# Autodesk Inventor assembly: 右足アセンブリ
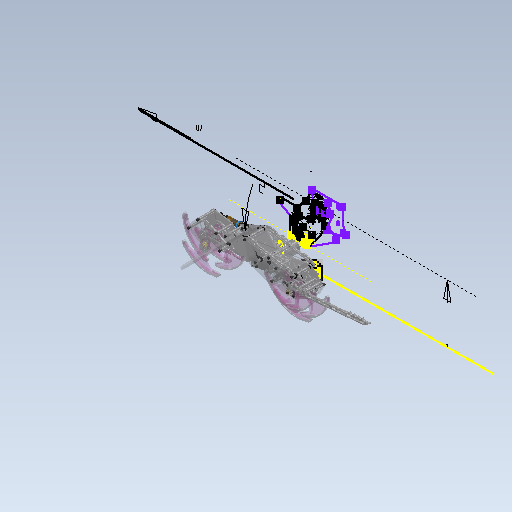
[picture p0: Inventor's stored thumbnail of the model, 512x512]
Saved by Autodesk Inventor 2020 (Build 240168000, 168)
## iProperties
Created: 2019-09-17
Part Number: 右足アセンブリ
Material: 一般
Document SubType Name: Assembly
Designer: tanjihayato
Mass: 847.137 g
Surface Area: 3618.61 cm^2
Volume: 359.726 cm^3
Density: 2.35495 g/cm^3
Author: tanjihayato
## Documents named in this file (54)
- \\Mac\Home\Documents\Inventor\2019お遊び機体\右足アセンブリ.iam
- \\Mac\Home\Documents\Inventor\2019お遊び機体\前足内フレーム.ipt
- \\Mac\Home\Documents\Inventor\2019お遊び機体\新型３クランクアセンブリ.iam
- \\Mac\Home\Documents\Inventor\2019お遊び機体\新型３脚最終段カム.ipt
- \\Mac\Home\Documents\Inventor\2019お遊び機体\スペーサ　m3-l35.ipt
- \\Mac\Home\Documents\Inventor\2019お遊び機体\新型３ヘッケン.ipt
- \\Mac\Home\Documents\Inventor\2019お遊び機体\新型３揺動節.ipt
- \\Mac\Home\Documents\Inventor\2019お遊び機体\線図.ipt
- \\Mac\Home\Documents\Inventor\2019お遊び機体\ギアトレイン.ipt
- \\Mac\Home\Documents\Inventor\2019お遊び機体\前足外フレーム.ipt
- \\Mac\Home\Documents\Inventor\2019お遊び機体\後ろ脚内フレーム.ipt
- \\Mac\Home\Documents\Inventor\2019お遊び機体\後ろ脚内フレーム２.ipt
- \\Mac\Home\Documents\Inventor\2019お遊び機体\新型３クランクアセンブリ_MIR.iam
- \\Mac\Home\Documents\Inventor\2019お遊び機体\新型３ヘッケン_MIR.ipt
- \\Mac\Home\Documents\Inventor\2019お遊び機体\新型３揺動節_MIR.ipt
- \\Mac\Home\Documents\Inventor\2019お遊び機体\後ろ脚外フレーム.ipt
- \\Mac\Home\Documents\Inventor\2019お遊び機体\前足ギアトレイン抑え.ipt
- \\Mac\Home\Documents\Inventor\2019お遊び機体\スペーサ　m3-l6.ipt
- \\Mac\Home\Documents\Inventor\2019お遊び機体\z28ギア(インベンター).ipt
- \\Mac\Home\Documents\Inventor\2019お遊び機体\z20ギア(インベンター).ipt
- \\Mac\Home\Documents\Inventor\2019お遊び機体\ベアリングフランジ6-12.ipt
- \\Mac\Home\Documents\Inventor\2019お遊び機体\z17ギア(インベンター).ipt
- \\Mac\Home\Documents\Inventor\2019お遊び機体\新型３脚最終段カム2.ipt
- \\Mac\Home\Documents\Inventor\2019お遊び機体\中間内フレーム2.ipt
- \\Mac\Home\Documents\Inventor\2019お遊び機体\サス軸抑え外.ipt
- \\Mac\Home\Documents\Inventor\2019お遊び機体\中間外フレーム2.ipt
- \\Mac\Home\Documents\Inventor\2019お遊び機体\タミヤダンパー1.iam
- \\Mac\Home\Documents\Inventor\2019お遊び機体\脚ゴム.ipt
- \\Mac\Home\Documents\Inventor\2019お遊び機体\歯車m0.5.z80.ipt
- \\Mac\Home\Documents\Inventor\2019お遊び機体\m2z10.ipt
- \\Mac\Home\Documents\Inventor\2019お遊び機体\中間フレーム内内.ipt
- \\Mac\Home\Documents\Inventor\2019お遊び機体\モーター(形だけ).ipt
- \\Mac\Home\Documents\Inventor\2019お遊び機体\脚モーターマウント.ipt
- \\Mac\Home\Documents\Inventor\2019お遊び機体\台形サスバー２.ipt
- \\Mac\Home\Documents\Inventor\2019お遊び機体\フランジブッシュ　d6-D8-l5-h12.ipt
- \\Mac\Home\Documents\Inventor\2019お遊び機体\スペーサ　m3-l45.ipt
- \\Mac\Home\Documents\Inventor\2019お遊び機体\台形サスバー板.ipt
- \\Mac\Home\Documents\Inventor\2019お遊び機体\台形サスカバー.ipt
- \\Mac\Home\Documents\Inventor\2019お遊び機体\カウンター短.ipt
- \\Mac\Home\Documents\Inventor\2019お遊び機体\ベアリングH　d6-D10-B3.ipt
- \\Mac\Home\Documents\Inventor\2019お遊び機体\スペーサ　m4-l35.ipt
- \\Mac\Home\Documents\Inventor\2019お遊び機体\スペーサ　m3-l14.ipt
- \\Mac\Home\Documents\Inventor\2019お遊び機体\キャップボルトM3×8.ipt
- \\Mac\Home\Documents\Inventor\2019お遊び機体\スペーサ　m3-l4.ipt
- \\Mac\Home\Documents\Inventor\2019お遊び機体\フランジブッシュ　d12-14-F20.ipt
- \\Mac\Home\Documents\Inventor\2019お遊び機体\オイレス　d12-D14-L3.ipt
- \\Mac\Home\Documents\Inventor\2019お遊び機体\キャップボルトM3×20.ipt
- \\Mac\Home\Documents\Inventor\2019お遊び機体\後ろ脚内内フレーム.ipt
- \\Mac\Home\Documents\Inventor\2019お遊び機体\ウイング土台.ipt
- \\Mac\Home\Documents\Inventor\2019お遊び機体\新型４ウイング.ipt
- \\Mac\Home\Documents\Inventor\2019お遊び機体\ウイング抑え.ipt
- \\Mac\Home\Documents\Inventor\2019お遊び機体\ねじ皿　m3-l8.ipt
- \\Mac\Home\Documents\Inventor\2019お遊び機体\新型４留め具.ipt
- \\Mac\Home\Documents\Inventor\2019お遊び機体\モーターマウントっぽい.ipt
## Components (192 placed, 53 different names)
1. 前足内フレーム:1 — 挿入:29, 挿入:32, 挿入:37, 挿入:127, 挿入:134, 挿入:135, 挿入:152, 挿入:181, 挿入:229, 挿入:230
2. 新型３クランクアセンブリ:1 [sub-assembly] — 挿入:1, メイト:1, 挿入:8, 挿入:9, 挿入:10, 挿入:11, 挿入:230
3. 新型３脚最終段カム:1 — 挿入:1, メイト:1, 挿入:62, メイト:44
4. スペーサ　m3-l35:2 — 挿入:29, 挿入:149
5. スペーサ　m3-l35:4 — メイト:2, メイト:3, メイト:4, メイト:5, 挿入:32, メイト:15
6. 新型３ヘッケン:1 — 挿入:11, 挿入:14, メイト:56, メイト:57, フラッシュ:2
7. 新型３ヘッケン:2 — 挿入:10, 挿入:13, メイト:60, メイト:61, フラッシュ:4
8. 新型３ヘッケン:3 — 挿入:9, 挿入:12, メイト:62, メイト:63, フラッシュ:5
9. 新型３ヘッケン:4 — 挿入:7, 挿入:8, メイト:58, メイト:59, フラッシュ:3
10. 新型３揺動節:1 — メイト:2, 挿入:7
11. 新型３揺動節:2 — メイト:3, 挿入:13
12. 新型３揺動節:3 — メイト:4, 挿入:12
13. 新型３揺動節:4 — メイト:5, 挿入:14
14. 線図:1 — メイト:91, メイト:92
15. ギアトレイン:1 — 挿入:15, 挿入:16, 挿入:17, 挿入:18, 挿入:19, 挿入:20, 挿入:154, 挿入:189
16. ギアトレイン:2 — 挿入:21, メイト:10, 挿入:37, 挿入:153, 挿入:187
17. スペーサ　m3-l6:3 — 挿入:17
18. スペーサ　m3-l6:2 — 挿入:20, メイト:10
19. スペーサ　m3-l6:5 — 挿入:19
20. スペーサ　m3-l6:1 — 挿入:16, 挿入:69
21. スペーサ　m3-l6:6 — 挿入:15, 挿入:21
22. スペーサ　m3-l6:4 — 挿入:18, 挿入:67
23. スペーサ　m3-l35:5 — メイト:55, 挿入:119
24. スペーサ　m3-l35:6
25. スペーサ　m3-l35:8 — メイト:53
26. 前足外フレーム:1 — メイト:15, 挿入:128, 挿入:136, メイト:84, 挿入:149, 挿入:165, 挿入:182, 挿入:226
27. 後ろ脚内フレーム:1 — 挿入:41, メイト:17, 挿入:71, 挿入:73, 挿入:76, 挿入:77, 挿入:188, 挿入:192, 挿入:193, 挿入:194, 挿入:195
28. 後ろ脚内フレーム２:1 — 挿入:41, メイト:17, 挿入:51, 挿入:52, 挿入:53, 挿入:54, 挿入:138, 挿入:139, 挿入:140, 挿入:155, 挿入:205, 挿入:227
29. 新型３クランクアセンブリ_MIR:1 [sub-assembly] — 挿入:43, 挿入:44, 挿入:45, 挿入:46, 挿入:55, メイト:18
30. 新型３ヘッケン_MIR:1 — 挿入:43, 挿入:50, メイト:66, メイト:67, フラッシュ:7
31. 新型３ヘッケン_MIR:2 — 挿入:44, 挿入:48, メイト:64, メイト:65, フラッシュ:6
32. 新型３ヘッケン_MIR:3 — 挿入:45, 挿入:49, メイト:68, メイト:69, フラッシュ:8
33. 新型３ヘッケン_MIR:4 — 挿入:46, 挿入:47, メイト:70, メイト:71, フラッシュ:9
34. 新型３揺動節_MIR:1 — 挿入:47, メイト:20
35. 新型３揺動節_MIR:3 — 挿入:49, メイト:21
36. 新型３揺動節_MIR:4 — 挿入:50, メイト:19
37. スペーサ　m3-l35:9 — 挿入:52, メイト:23
38. スペーサ　m3-l35:10 — 挿入:51
39. スペーサ　m3-l35:11 — 挿入:54, メイト:19, メイト:20, メイト:21, メイト:22, 挿入:57
40. スペーサ　m3-l35:12 — 挿入:53
41. 新型３脚最終段カム:2 — 挿入:55, メイト:18, 挿入:74, メイト:48, 挿入:227
42. 後ろ脚外フレーム:1 — 挿入:57, メイト:23, 挿入:141, 挿入:142, 挿入:143, 挿入:144, 挿入:225
43. 前足ギアトレイン抑え:1 — 挿入:151, 挿入:237, 挿入:238, 挿入:239, 挿入:240
44. スペーサ　m3-l14:1
45. スペーサ　m3-l14:2 — 挿入:237
46. スペーサ　m3-l14:3 — 挿入:229
47. 新型３脚最終段カム2:1 — 挿入:62, メイト:44, 挿入:63, メイト:45
48. z28ギア(インベンター):1 — 挿入:63, メイト:45, 挿入:64, メイト:47
49. 新型３脚最終段カム:4 — 挿入:65, メイト:46, メイト:100
50. 新型３脚最終段カム:5 — 挿入:64, 挿入:65, メイト:46, メイト:47
51. z20ギア(インベンター):1 — 挿入:66
52. ベアリングフランジ6-12:1 — 挿入:66, 挿入:67
53. z17ギア(インベンター):1 — 挿入:68
54. ベアリングフランジ6-12:2 — 挿入:68, 挿入:69
55. z17ギア(インベンター):2
56. ベアリングフランジ6-12:3 — 挿入:71
57. z20ギア(インベンター):2
58. ベアリングフランジ6-12:4 — 挿入:73
59. z28ギア(インベンター):2 — 挿入:75, メイト:49
60. 新型３脚最終段カム:6 — 挿入:74, メイト:48, 挿入:75, メイト:49
61. スペーサ　m3-l6:7 — 挿入:76
62. スペーサ　m3-l6:8 — 挿入:77
63. 中間内フレーム2:1 — 挿入:78, メイト:50, 挿入:94, 挿入:95, 挿入:96, 挿入:97, 挿入:98, 挿入:124, 挿入:147, 挿入:148, 挿入:217, 挿入:218, 挿入:221, 挿入:231, 挿入:232, 挿入:233, 挿入:234, 挿入:235, 挿入:236
64. サス軸抑え外:1 — 挿入:78, メイト:50, 挿入:198, 挿入:199, 挿入:200, 挿入:201
65. 中間外フレーム2:1 — メイト:53, 挿入:119, メイト:79, 挿入:120, 挿入:145, 挿入:146, 挿入:164, 挿入:213, メイト:88, 挿入:219, 挿入:220, メイト:91, メイト:92
66. スペーサ　m3-l4:2
67. スペーサ　m3-l4:1
68. スペーサ　m3-l4:3
69. タミヤダンパー1:1 [sub-assembly] — メイト:55, 挿入:118
70. 脚ゴム:1 — メイト:68, メイト:69, フラッシュ:8
71. 脚ゴム:2 — メイト:70, メイト:71, フラッシュ:9
72. 脚ゴム:3 — メイト:56, メイト:57, フラッシュ:2
73. 脚ゴム:4 — メイト:66, メイト:67, フラッシュ:7
74. 脚ゴム:5 — メイト:60, メイト:61, フラッシュ:4
75. 脚ゴム:6 — メイト:64, メイト:65, フラッシュ:6
76. 脚ゴム:7 — メイト:62, メイト:63, フラッシュ:5
77. 脚ゴム:8 — メイト:58, メイト:59, フラッシュ:3
78. 歯車m0.5.z80:1 — 挿入:102, 挿入:103, 挿入:104, 挿入:105, メイト:74
79. m2z10:1 — 挿入:94, 挿入:106, メイト:74
80. スペーサ　m3-l6:9 — 挿入:98, メイト:73, メイト:75
81. スペーサ　m3-l6:10 — 挿入:96
82. スペーサ　m3-l6:11 — 挿入:95
83. スペーサ　m3-l6:12 — 挿入:97, 挿入:99, 挿入:107
84. サス軸抑え外:2 — 挿入:99, メイト:73, 挿入:183, 挿入:184, 挿入:185, 挿入:186, 挿入:202, 挿入:203
85. スペーサ　m3-l6:13 — 挿入:105
86. スペーサ　m3-l6:14 — 挿入:104
87. スペーサ　m3-l6:15 — 挿入:103
88. スペーサ　m3-l6:16 — 挿入:102, 挿入:106
89. 中間フレーム内内:1 — 挿入:107, メイト:75, 挿入:172, 挿入:173, 挿入:208, 挿入:209, 挿入:210, 挿入:211
90. モーター(形だけ):1 — 挿入:242
91. モーター(形だけ):2 — 挿入:243
92. スペーサ　m3-l14:6 — 挿入:211, 挿入:212
93. スペーサ　m3-l14:4 — 挿入:209
94. スペーサ　m3-l14:5 — 挿入:210
95. スペーサ　m3-l14:7 — 挿入:208, メイト:87
96. 脚モーターマウント:1 — 挿入:166, 挿入:167, 挿入:168, 挿入:169, 挿入:212, メイト:93, メイト:94, メイト:95, メイト:96, メイト:97, メイト:98, 挿入:228
97. 台形サスバー２:1 — メイト:79, 挿入:121, 挿入:122, 挿入:123, 挿入:129, 挿入:130, メイト:83, 挿入:160
98. 台形サスバー２:2 — 挿入:118, メイト:81, フラッシュ:10, メイト:82, 挿入:137, メイト:85, 挿入:156, 挿入:157, 挿入:158, 挿入:159
99. フランジブッシュ　d6-D8-l5-h12:1 — 挿入:128, 挿入:150
100. フランジブッシュ　d6-D8-l5-h12:2 — 挿入:120
101. フランジブッシュ　d6-D8-l5-h12:3 — 挿入:127
102. フランジブッシュ　d6-D8-l5-h12:4 — 挿入:124, 挿入:137
103. スペーサ　m3-l45:1 — 挿入:121
104. スペーサ　m3-l45:2 — 挿入:122, メイト:85, 挿入:150
105. スペーサ　m3-l45:3 — 挿入:123
106. スペーサ　m3-l45:4 — 挿入:129
107. 台形サスバー板:1 — メイト:81, フラッシュ:10, メイト:82
108. 台形サスカバー:1 — 挿入:130, メイト:83, 挿入:161, 挿入:162, 挿入:163
109. カウンター短:1 — 挿入:136, メイト:84
110. ベアリングH　d6-D10-B3:1 — 挿入:225
111. ベアリングH　d6-D10-B3:2 — 挿入:226
112. スペーサ　m4-l35:1 — 挿入:135
113. スペーサ　m4-l35:2 — 挿入:134
114. キャップボルトM3×8:1 — 挿入:138
115. キャップボルトM3×8:2 — 挿入:139
116. キャップボルトM3×8:3 — 挿入:141
117. キャップボルトM3×8:4 — 挿入:144
118. キャップボルトM3×8:5 — 挿入:140
119. キャップボルトM3×8:6 — 挿入:145
120. キャップボルトM3×8:7 — 挿入:146
121. キャップボルトM3×8:8 — 挿入:143
122. キャップボルトM3×8:9 — 挿入:142
123. キャップボルトM3×8:10 — 挿入:147
124. キャップボルトM3×8:11 — 挿入:148
125. フランジブッシュ　d12-14-F20:1 — 挿入:151, メイト:100
126. フランジブッシュ　d12-14-F20:2 — 挿入:152
127. フランジブッシュ　d12-14-F20:3 — 挿入:155
128. オイレス　d12-D14-L3:1 — 挿入:153
129. オイレス　d12-D14-L3:2 — 挿入:154
130. キャップボルトM3×8:12 — 挿入:156
131. キャップボルトM3×8:13 — 挿入:157
132. キャップボルトM3×8:14 — 挿入:160
133. キャップボルトM3×8:15 — 挿入:159
134. キャップボルトM3×8:16 — 挿入:161
135. キャップボルトM3×8:17 — 挿入:162
136. キャップボルトM3×8:18 — 挿入:158
137. キャップボルトM3×8:19 — 挿入:163
138. キャップボルトM3×8:20 — 挿入:164
139. キャップボルトM3×8:21 — 挿入:166, メイト:87
140. キャップボルトM3×8:22 — 挿入:165
141. キャップボルトM3×8:23 — 挿入:167, 挿入:241
142. キャップボルトM3×8:24 — 挿入:168
143. キャップボルトM3×8:25 — 挿入:169, メイト:102
144. キャップボルトM3×8:26 — 挿入:236
145. キャップボルトM3×8:27 — 挿入:235
146. キャップボルトM3×8:30 — 挿入:172
147. キャップボルトM3×8:31 — 挿入:173
148. キャップボルトM3×20:1 — 挿入:239
149. キャップボルトM3×20:2 — 挿入:238
150. キャップボルトM3×20:3 — 挿入:240
151. キャップボルトM3×20:4 — 挿入:184
152. キャップボルトM3×20:5 — 挿入:183
153. キャップボルトM3×20:6 — 挿入:185
154. キャップボルトM3×20:7 — 挿入:186
155. キャップボルトM3×8:32 — 挿入:181
156. キャップボルトM3×8:33 — 挿入:182
157. スペーサ　m3-l4:4 — 挿入:187, 挿入:196, 挿入:199
158. スペーサ　m3-l4:5 — 挿入:188, 挿入:197, 挿入:198
159. スペーサ　m3-l4:6 — 挿入:189
160. キャップボルトM3×20:8 — 挿入:196
161. キャップボルトM3×20:9 — 挿入:197
162. スペーサ　m3-l6:17 — 挿入:195
163. スペーサ　m3-l6:18 — 挿入:194
164. スペーサ　m3-l6:19 — 挿入:193, 挿入:204
165. スペーサ　m3-l6:20 — 挿入:192, メイト:86
166. フランジブッシュ　d6-D8-l5-h12:5 — 挿入:202
167. フランジブッシュ　d6-D8-l5-h12:6 — 挿入:203
168. フランジブッシュ　d6-D8-l5-h12:7 — 挿入:200
169. フランジブッシュ　d6-D8-l5-h12:8 — 挿入:201
170. 後ろ脚内内フレーム:1 — 挿入:204, メイト:86, メイト:99
171. キャップボルトM3×8:34 — 挿入:205
172. ウイング土台:1 — 挿入:213, メイト:88, 挿入:214, 挿入:215, メイト:89
173. スペーサ　m3-l6:21 — 挿入:214, メイト:90
174. スペーサ　m3-l6:22 — 挿入:215, 挿入:224, メイト:101
175. 新型４ウイング:1 — メイト:89, メイト:101
176. ウイング抑え:1 — 挿入:222, 挿入:223, 挿入:224
177. ねじ皿　m3-l8:1 — 挿入:217
178. ねじ皿　m3-l8:2 — 挿入:218
179. ねじ皿　m3-l8:3 — 挿入:219
180. ねじ皿　m3-l8:4 — 挿入:221
181. ねじ皿　m3-l8:5 — 挿入:220
182. キャップボルトM3×8:35 — 挿入:222
183. キャップボルトM3×8:36 — 挿入:223, メイト:90
184. 新型４留め具:1 — メイト:94, メイト:95, メイト:98
185. 新型４留め具:4 — メイト:93, メイト:96, メイト:97
186. タミヤダンパー1:2 [sub-assembly] — 挿入:228, メイト:99
187. スペーサ　m3-l6:23 — 挿入:232
188. スペーサ　m3-l6:24 — 挿入:231
189. スペーサ　m3-l6:25 — 挿入:234
190. スペーサ　m3-l6:26 — 挿入:233
191. モーターマウントっぽい:1 — 挿入:241, メイト:102, 挿入:242, 挿入:243
192. 新型３揺動節_MIR:2 — 挿入:48, メイト:22
## Relationships (252: Insert 178, Mate 65, Flush 9)
- 挿入:1 [Insert]: 新型３クランクアセンブリ:1 ↔ 新型３脚最終段カム:1
- メイト:1 [Mate]: 新型３クランクアセンブリ:1 ↔ 新型３脚最終段カム:1
- メイト:2 [Mate]: スペーサ　m3-l35:4 ↔ 新型３揺動節:1
- メイト:3 [Mate]: スペーサ　m3-l35:4 ↔ 新型３揺動節:2
- メイト:4 [Mate]: スペーサ　m3-l35:4 ↔ 新型３揺動節:3
- メイト:5 [Mate]: スペーサ　m3-l35:4 ↔ 新型３揺動節:4
- 挿入:7 [Insert]: 新型３ヘッケン:4 ↔ 新型３揺動節:1
- 挿入:8 [Insert] (0.25 mm): 新型３クランクアセンブリ:1 ↔ 新型３ヘッケン:4
- 挿入:9 [Insert] (0.25 mm): 新型３クランクアセンブリ:1 ↔ 新型３ヘッケン:3
- 挿入:10 [Insert] (0.25 mm): 新型３クランクアセンブリ:1 ↔ 新型３ヘッケン:2
- 挿入:11 [Insert] (0.25 mm): 新型３クランクアセンブリ:1 ↔ 新型３ヘッケン:1
- 挿入:12 [Insert]: 新型３ヘッケン:3 ↔ 新型３揺動節:3
- 挿入:13 [Insert]: 新型３ヘッケン:2 ↔ 新型３揺動節:2
- 挿入:14 [Insert]: 新型３ヘッケン:1 ↔ 新型３揺動節:4
- 挿入:15 [Insert]: ギアトレイン:1 ↔ スペーサ　m3-l6:6
- 挿入:16 [Insert]: ギアトレイン:1 ↔ スペーサ　m3-l6:1
- 挿入:17 [Insert]: ギアトレイン:1 ↔ スペーサ　m3-l6:3
- 挿入:18 [Insert]: ギアトレイン:1 ↔ スペーサ　m3-l6:4
- 挿入:19 [Insert]: ギアトレイン:1 ↔ スペーサ　m3-l6:5
- 挿入:20 [Insert]: ギアトレイン:1 ↔ スペーサ　m3-l6:2
- 挿入:21 [Insert]: ギアトレイン:2 ↔ スペーサ　m3-l6:6
- メイト:10 [Mate]: ギアトレイン:2 ↔ スペーサ　m3-l6:2
- 挿入:29 [Insert]: 前足内フレーム:1 ↔ スペーサ　m3-l35:2
- 挿入:32 [Insert]: 前足内フレーム:1 ↔ スペーサ　m3-l35:4
- 挿入:37 [Insert] (1 mm): 前足内フレーム:1 ↔ ギアトレイン:2
- メイト:15 [Mate]: スペーサ　m3-l35:4 ↔ 前足外フレーム:1
- 挿入:41 [Insert]: 後ろ脚内フレーム:1 ↔ 後ろ脚内フレーム２:1
- メイト:17 [Mate]: 後ろ脚内フレーム:1 ↔ 後ろ脚内フレーム２:1
- 挿入:43 [Insert] (0.25 mm): 新型３クランクアセンブリ_MIR:1 ↔ 新型３ヘッケン_MIR:1
- 挿入:44 [Insert] (0.25 mm): 新型３クランクアセンブリ_MIR:1 ↔ 新型３ヘッケン_MIR:2
- 挿入:45 [Insert] (0.25 mm): 新型３クランクアセンブリ_MIR:1 ↔ 新型３ヘッケン_MIR:3
- 挿入:46 [Insert] (0.25 mm): 新型３クランクアセンブリ_MIR:1 ↔ 新型３ヘッケン_MIR:4
- 挿入:47 [Insert]: 新型３ヘッケン_MIR:4 ↔ 新型３揺動節_MIR:1
- 挿入:48 [Insert]: 新型３ヘッケン_MIR:2 ↔ 新型３揺動節_MIR:2
- 挿入:49 [Insert]: 新型３ヘッケン_MIR:3 ↔ 新型３揺動節_MIR:3
- 挿入:50 [Insert]: 新型３ヘッケン_MIR:1 ↔ 新型３揺動節_MIR:4
- 挿入:51 [Insert]: 後ろ脚内フレーム２:1 ↔ スペーサ　m3-l35:10
- 挿入:52 [Insert]: 後ろ脚内フレーム２:1 ↔ スペーサ　m3-l35:9
- 挿入:53 [Insert]: 後ろ脚内フレーム２:1 ↔ スペーサ　m3-l35:12
- 挿入:54 [Insert]: 後ろ脚内フレーム２:1 ↔ スペーサ　m3-l35:11
- 挿入:55 [Insert]: 新型３クランクアセンブリ_MIR:1 ↔ 新型３脚最終段カム:2
- メイト:18 [Mate]: 新型３クランクアセンブリ_MIR:1 ↔ 新型３脚最終段カム:2
- メイト:19 [Mate]: 新型３揺動節_MIR:4 ↔ スペーサ　m3-l35:11
- メイト:20 [Mate]: 新型３揺動節_MIR:1 ↔ スペーサ　m3-l35:11
- メイト:21 [Mate]: 新型３揺動節_MIR:3 ↔ スペーサ　m3-l35:11
- メイト:22 [Mate]: スペーサ　m3-l35:11 ↔ 新型３揺動節_MIR:2
- 挿入:57 [Insert]: スペーサ　m3-l35:11 ↔ 後ろ脚外フレーム:1
- メイト:23 [Mate]: スペーサ　m3-l35:9 ↔ 後ろ脚外フレーム:1
- [Insert]: 前足内フレーム:1 ↔ スペーサ　m3-l14:2
- [Insert]: 前足内フレーム:1 ↔ スペーサ　m3-l14:1
- 挿入:62 [Insert]: 新型３脚最終段カム:1 ↔ 新型３脚最終段カム2:1
- メイト:44 [Mate]: 新型３脚最終段カム:1 ↔ 新型３脚最終段カム2:1
- 挿入:63 [Insert]: 新型３脚最終段カム2:1 ↔ z28ギア(インベンター):1
- メイト:45 [Mate]: 新型３脚最終段カム2:1 ↔ z28ギア(インベンター):1
- 挿入:64 [Insert]: z28ギア(インベンター):1 ↔ 新型３脚最終段カム:5
- 挿入:65 [Insert]: 新型３脚最終段カム:4 ↔ 新型３脚最終段カム:5
- メイト:46 [Mate]: 新型３脚最終段カム:4 ↔ 新型３脚最終段カム:5
- メイト:47 [Mate]: z28ギア(インベンター):1 ↔ 新型３脚最終段カム:5
- 挿入:66 [Insert]: z20ギア(インベンター):1 ↔ ベアリングフランジ6-12:1
- 挿入:67 [Insert] (1 mm): スペーサ　m3-l6:4 ↔ ベアリングフランジ6-12:1
- 挿入:68 [Insert]: z17ギア(インベンター):1 ↔ ベアリングフランジ6-12:2
- 挿入:69 [Insert] (1 mm): スペーサ　m3-l6:1 ↔ ベアリングフランジ6-12:2
- [Insert]: z17ギア(インベンター):2 ↔ ベアリングフランジ6-12:3
- 挿入:71 [Insert] (1 mm): 後ろ脚内フレーム:1 ↔ ベアリングフランジ6-12:3
- [Insert]: z20ギア(インベンター):2 ↔ ベアリングフランジ6-12:4
- 挿入:73 [Insert] (1 mm): 後ろ脚内フレーム:1 ↔ ベアリングフランジ6-12:4
- 挿入:74 [Insert]: 新型３脚最終段カム:2 ↔ 新型３脚最終段カム:6
- メイト:48 [Mate]: 新型３脚最終段カム:2 ↔ 新型３脚最終段カム:6
- 挿入:75 [Insert]: z28ギア(インベンター):2 ↔ 新型３脚最終段カム:6
- メイト:49 [Mate]: z28ギア(インベンター):2 ↔ 新型３脚最終段カム:6
- 挿入:76 [Insert]: 後ろ脚内フレーム:1 ↔ スペーサ　m3-l6:7
- 挿入:77 [Insert]: 後ろ脚内フレーム:1 ↔ スペーサ　m3-l6:8
- 挿入:78 [Insert] (1 mm): 中間内フレーム2:1 ↔ サス軸抑え外:1
- メイト:50 [Mate]: 中間内フレーム2:1 ↔ サス軸抑え外:1
- メイト:53 [Mate]: スペーサ　m3-l35:8 ↔ 中間外フレーム2:1
- [Insert]: スペーサ　m3-l35:6 ↔ スペーサ　m3-l4:2
- [Insert]: スペーサ　m3-l35:8 ↔ スペーサ　m3-l4:3
- [Insert]: スペーサ　m3-l35:5 ↔ スペーサ　m3-l4:1
- [Insert]: 中間内フレーム2:1 ↔ スペーサ　m3-l4:3
- [Insert]: 中間内フレーム2:1 ↔ スペーサ　m3-l4:2
- [Insert]: 中間内フレーム2:1 ↔ スペーサ　m3-l4:1
- メイト:55 [Mate]: スペーサ　m3-l35:5 ↔ タミヤダンパー1:1
- メイト:56 [Mate]: 新型３ヘッケン:1 ↔ 脚ゴム:3
- メイト:57 [Mate]: 新型３ヘッケン:1 ↔ 脚ゴム:3
- フラッシュ:2 [Flush]: 新型３ヘッケン:1 ↔ 脚ゴム:3
- メイト:58 [Mate]: 新型３ヘッケン:4 ↔ 脚ゴム:8
- メイト:59 [Mate]: 新型３ヘッケン:4 ↔ 脚ゴム:8
- フラッシュ:3 [Flush]: 新型３ヘッケン:4 ↔ 脚ゴム:8
- メイト:60 [Mate]: 新型３ヘッケン:2 ↔ 脚ゴム:5
- メイト:61 [Mate]: 新型３ヘッケン:2 ↔ 脚ゴム:5
- フラッシュ:4 [Flush]: 新型３ヘッケン:2 ↔ 脚ゴム:5
- メイト:62 [Mate]: 新型３ヘッケン:3 ↔ 脚ゴム:7
- メイト:63 [Mate]: 新型３ヘッケン:3 ↔ 脚ゴム:7
- フラッシュ:5 [Flush]: 新型３ヘッケン:3 ↔ 脚ゴム:7
- メイト:64 [Mate]: 新型３ヘッケン_MIR:2 ↔ 脚ゴム:6
- メイト:65 [Mate]: 新型３ヘッケン_MIR:2 ↔ 脚ゴム:6
- フラッシュ:6 [Flush]: 新型３ヘッケン_MIR:2 ↔ 脚ゴム:6
- メイト:66 [Mate]: 新型３ヘッケン_MIR:1 ↔ 脚ゴム:4
- メイト:67 [Mate]: 新型３ヘッケン_MIR:1 ↔ 脚ゴム:4
- フラッシュ:7 [Flush]: 新型３ヘッケン_MIR:1 ↔ 脚ゴム:4
- メイト:68 [Mate]: 新型３ヘッケン_MIR:3 ↔ 脚ゴム:1
- メイト:69 [Mate]: 新型３ヘッケン_MIR:3 ↔ 脚ゴム:1
- フラッシュ:8 [Flush]: 新型３ヘッケン_MIR:3 ↔ 脚ゴム:1
- メイト:70 [Mate]: 新型３ヘッケン_MIR:4 ↔ 脚ゴム:2
- メイト:71 [Mate]: 新型３ヘッケン_MIR:4 ↔ 脚ゴム:2
- フラッシュ:9 [Flush]: 新型３ヘッケン_MIR:4 ↔ 脚ゴム:2
- 挿入:94 [Insert] (0.5 mm): 中間内フレーム2:1 ↔ m2z10:1
- 挿入:95 [Insert]: 中間内フレーム2:1 ↔ スペーサ　m3-l6:11
- 挿入:96 [Insert]: 中間内フレーム2:1 ↔ スペーサ　m3-l6:10
- 挿入:97 [Insert]: 中間内フレーム2:1 ↔ スペーサ　m3-l6:12
- 挿入:98 [Insert]: 中間内フレーム2:1 ↔ スペーサ　m3-l6:9
- 挿入:99 [Insert] (4 mm): スペーサ　m3-l6:12 ↔ サス軸抑え外:2
- メイト:73 [Mate]: スペーサ　m3-l6:9 ↔ サス軸抑え外:2
- 挿入:102 [Insert]: 歯車m0.5.z80:1 ↔ スペーサ　m3-l6:16
- 挿入:103 [Insert]: 歯車m0.5.z80:1 ↔ スペーサ　m3-l6:15
- 挿入:104 [Insert]: 歯車m0.5.z80:1 ↔ スペーサ　m3-l6:14
- 挿入:105 [Insert]: 歯車m0.5.z80:1 ↔ スペーサ　m3-l6:13
- 挿入:106 [Insert]: m2z10:1 ↔ スペーサ　m3-l6:16
- メイト:74 [Mate]: 歯車m0.5.z80:1 ↔ m2z10:1
- 挿入:107 [Insert]: スペーサ　m3-l6:12 ↔ 中間フレーム内内:1
- メイト:75 [Mate]: スペーサ　m3-l6:9 ↔ 中間フレーム内内:1
- 挿入:118 [Insert] (30 mm): タミヤダンパー1:1 ↔ 台形サスバー２:2
- 挿入:119 [Insert]: スペーサ　m3-l35:5 ↔ 中間外フレーム2:1
- メイト:79 [Mate]: 中間外フレーム2:1 ↔ 台形サスバー２:1
- 挿入:120 [Insert]: 中間外フレーム2:1 ↔ フランジブッシュ　d6-D8-l5-h12:2
- 挿入:121 [Insert]: 台形サスバー２:1 ↔ スペーサ　m3-l45:1
- 挿入:122 [Insert]: 台形サスバー２:1 ↔ スペーサ　m3-l45:2
- 挿入:123 [Insert]: 台形サスバー２:1 ↔ スペーサ　m3-l45:3
- 挿入:124 [Insert]: 中間内フレーム2:1 ↔ フランジブッシュ　d6-D8-l5-h12:4
- 挿入:127 [Insert]: 前足内フレーム:1 ↔ フランジブッシュ　d6-D8-l5-h12:3
- 挿入:128 [Insert]: 前足外フレーム:1 ↔ フランジブッシュ　d6-D8-l5-h12:1
- 挿入:129 [Insert]: 台形サスバー２:1 ↔ スペーサ　m3-l45:4
- メイト:81 [Mate]: 台形サスバー２:2 ↔ 台形サスバー板:1
- フラッシュ:10 [Flush]: 台形サスバー２:2 ↔ 台形サスバー板:1
- メイト:82 [Mate]: 台形サスバー２:2 ↔ 台形サスバー板:1
- 挿入:130 [Insert]: 台形サスバー２:1 ↔ 台形サスカバー:1
- メイト:83 [Mate]: 台形サスバー２:1 ↔ 台形サスカバー:1
- 挿入:134 [Insert]: 前足内フレーム:1 ↔ スペーサ　m4-l35:2
- 挿入:135 [Insert]: 前足内フレーム:1 ↔ スペーサ　m4-l35:1
- 挿入:136 [Insert]: 前足外フレーム:1 ↔ カウンター短:1
- メイト:84 [Mate]: 前足外フレーム:1 ↔ カウンター短:1
- 挿入:137 [Insert]: 台形サスバー２:2 ↔ フランジブッシュ　d6-D8-l5-h12:4
- メイト:85 [Mate]: 台形サスバー２:2 ↔ スペーサ　m3-l45:2
- 挿入:138 [Insert]: 後ろ脚内フレーム２:1 ↔ キャップボルトM3×8:1
- 挿入:139 [Insert]: 後ろ脚内フレーム２:1 ↔ キャップボルトM3×8:2
- 挿入:140 [Insert]: 後ろ脚内フレーム２:1 ↔ キャップボルトM3×8:5
- 挿入:141 [Insert]: 後ろ脚外フレーム:1 ↔ キャップボルトM3×8:3
- 挿入:142 [Insert]: 後ろ脚外フレーム:1 ↔ キャップボルトM3×8:9
- 挿入:143 [Insert]: 後ろ脚外フレーム:1 ↔ キャップボルトM3×8:8
- 挿入:144 [Insert]: 後ろ脚外フレーム:1 ↔ キャップボルトM3×8:4
- 挿入:145 [Insert]: 中間外フレーム2:1 ↔ キャップボルトM3×8:6
- 挿入:146 [Insert]: 中間外フレーム2:1 ↔ キャップボルトM3×8:7
- 挿入:147 [Insert]: 中間内フレーム2:1 ↔ キャップボルトM3×8:10
- 挿入:148 [Insert]: 中間内フレーム2:1 ↔ キャップボルトM3×8:11
- 挿入:149 [Insert]: スペーサ　m3-l35:2 ↔ 前足外フレーム:1
- 挿入:150 [Insert]: フランジブッシュ　d6-D8-l5-h12:1 ↔ スペーサ　m3-l45:2
- 挿入:151 [Insert]: 前足ギアトレイン抑え:1 ↔ フランジブッシュ　d12-14-F20:1
- 挿入:152 [Insert]: 前足内フレーム:1 ↔ フランジブッシュ　d12-14-F20:2
- 挿入:153 [Insert]: ギアトレイン:2 ↔ オイレス　d12-D14-L3:1
- 挿入:154 [Insert]: ギアトレイン:1 ↔ オイレス　d12-D14-L3:2
- 挿入:155 [Insert]: 後ろ脚内フレーム２:1 ↔ フランジブッシュ　d12-14-F20:3
- 挿入:156 [Insert]: 台形サスバー２:2 ↔ キャップボルトM3×8:12
- 挿入:157 [Insert]: 台形サスバー２:2 ↔ キャップボルトM3×8:13
- 挿入:158 [Insert]: 台形サスバー２:2 ↔ キャップボルトM3×8:18
- 挿入:159 [Insert]: 台形サスバー２:2 ↔ キャップボルトM3×8:15
- 挿入:160 [Insert]: 台形サスバー２:1 ↔ キャップボルトM3×8:14
- 挿入:161 [Insert]: 台形サスカバー:1 ↔ キャップボルトM3×8:16
- 挿入:162 [Insert]: 台形サスカバー:1 ↔ キャップボルトM3×8:17
- 挿入:163 [Insert]: 台形サスカバー:1 ↔ キャップボルトM3×8:19
- 挿入:164 [Insert]: 中間外フレーム2:1 ↔ キャップボルトM3×8:20
- 挿入:165 [Insert]: 前足外フレーム:1 ↔ キャップボルトM3×8:22
- 挿入:166 [Insert]: 脚モーターマウント:1 ↔ キャップボルトM3×8:21
- 挿入:167 [Insert]: 脚モーターマウント:1 ↔ キャップボルトM3×8:23
- 挿入:168 [Insert]: 脚モーターマウント:1 ↔ キャップボルトM3×8:24
- 挿入:169 [Insert]: 脚モーターマウント:1 ↔ キャップボルトM3×8:25
- 挿入:172 [Insert]: 中間フレーム内内:1 ↔ キャップボルトM3×8:30
- 挿入:173 [Insert]: 中間フレーム内内:1 ↔ キャップボルトM3×8:31
- 挿入:181 [Insert]: 前足内フレーム:1 ↔ キャップボルトM3×8:32
- 挿入:182 [Insert]: 前足外フレーム:1 ↔ キャップボルトM3×8:33
- 挿入:183 [Insert]: サス軸抑え外:2 ↔ キャップボルトM3×20:5
- 挿入:184 [Insert]: サス軸抑え外:2 ↔ キャップボルトM3×20:4
- 挿入:185 [Insert]: サス軸抑え外:2 ↔ キャップボルトM3×20:6
- 挿入:186 [Insert]: サス軸抑え外:2 ↔ キャップボルトM3×20:7
- 挿入:187 [Insert]: ギアトレイン:2 ↔ スペーサ　m3-l4:4
- 挿入:188 [Insert]: 後ろ脚内フレーム:1 ↔ スペーサ　m3-l4:5
- 挿入:189 [Insert]: ギアトレイン:1 ↔ スペーサ　m3-l4:6
- 挿入:192 [Insert]: 後ろ脚内フレーム:1 ↔ スペーサ　m3-l6:20
- 挿入:193 [Insert]: 後ろ脚内フレーム:1 ↔ スペーサ　m3-l6:19
- 挿入:194 [Insert]: 後ろ脚内フレーム:1 ↔ スペーサ　m3-l6:18
- 挿入:195 [Insert]: 後ろ脚内フレーム:1 ↔ スペーサ　m3-l6:17
- 挿入:196 [Insert]: スペーサ　m3-l4:4 ↔ キャップボルトM3×20:8
- 挿入:197 [Insert]: スペーサ　m3-l4:5 ↔ キャップボルトM3×20:9
- 挿入:198 [Insert] (1 mm): サス軸抑え外:1 ↔ スペーサ　m3-l4:5
- 挿入:199 [Insert] (1 mm): サス軸抑え外:1 ↔ スペーサ　m3-l4:4
- 挿入:200 [Insert]: サス軸抑え外:1 ↔ フランジブッシュ　d6-D8-l5-h12:7
- 挿入:201 [Insert]: サス軸抑え外:1 ↔ フランジブッシュ　d6-D8-l5-h12:8
- 挿入:202 [Insert]: サス軸抑え外:2 ↔ フランジブッシュ　d6-D8-l5-h12:5
- 挿入:203 [Insert]: サス軸抑え外:2 ↔ フランジブッシュ　d6-D8-l5-h12:6
- 挿入:204 [Insert]: スペーサ　m3-l6:19 ↔ 後ろ脚内内フレーム:1
- メイト:86 [Mate]: スペーサ　m3-l6:20 ↔ 後ろ脚内内フレーム:1
- 挿入:205 [Insert]: 後ろ脚内フレーム２:1 ↔ キャップボルトM3×8:34
- 挿入:208 [Insert]: 中間フレーム内内:1 ↔ スペーサ　m3-l14:7
- 挿入:209 [Insert]: 中間フレーム内内:1 ↔ スペーサ　m3-l14:4
- 挿入:210 [Insert]: 中間フレーム内内:1 ↔ スペーサ　m3-l14:5
- 挿入:211 [Insert]: 中間フレーム内内:1 ↔ スペーサ　m3-l14:6
- 挿入:212 [Insert]: スペーサ　m3-l14:6 ↔ 脚モーターマウント:1
- メイト:87 [Mate]: スペーサ　m3-l14:7 ↔ キャップボルトM3×8:21
- 挿入:213 [Insert]: 中間外フレーム2:1 ↔ ウイング土台:1
- メイト:88 [Mate]: 中間外フレーム2:1 ↔ ウイング土台:1
- 挿入:214 [Insert]: ウイング土台:1 ↔ スペーサ　m3-l6:21
- 挿入:215 [Insert]: ウイング土台:1 ↔ スペーサ　m3-l6:22
- メイト:89 [Mate]: ウイング土台:1 ↔ 新型４ウイング:1
- 挿入:217 [Insert]: 中間内フレーム2:1 ↔ ねじ皿　m3-l8:1
- 挿入:218 [Insert]: 中間内フレーム2:1 ↔ ねじ皿　m3-l8:2
- 挿入:219 [Insert]: 中間外フレーム2:1 ↔ ねじ皿　m3-l8:3
- 挿入:220 [Insert]: 中間外フレーム2:1 ↔ ねじ皿　m3-l8:5
- 挿入:221 [Insert]: 中間内フレーム2:1 ↔ ねじ皿　m3-l8:4
- 挿入:222 [Insert]: ウイング抑え:1 ↔ キャップボルトM3×8:35
- 挿入:223 [Insert]: ウイング抑え:1 ↔ キャップボルトM3×8:36
- 挿入:224 [Insert]: スペーサ　m3-l6:22 ↔ ウイング抑え:1
- メイト:90 [Mate]: スペーサ　m3-l6:21 ↔ キャップボルトM3×8:36
- メイト:91 [Mate]: 線図:1 ↔ 中間外フレーム2:1
- メイト:92 [Mate] (-150 mm): 線図:1 ↔ 中間外フレーム2:1
- メイト:93 [Mate]: 脚モーターマウント:1 ↔ 新型４留め具:4
- メイト:94 [Mate]: 脚モーターマウント:1 ↔ 新型４留め具:1
- メイト:95 [Mate]: 脚モーターマウント:1 ↔ 新型４留め具:1
- メイト:96 [Mate]: 脚モーターマウント:1 ↔ 新型４留め具:4
- メイト:97 [Mate]: 脚モーターマウント:1 ↔ 新型４留め具:4
- メイト:98 [Mate]: 脚モーターマウント:1 ↔ 新型４留め具:1
- 挿入:225 [Insert]: 後ろ脚外フレーム:1 ↔ ベアリングH　d6-D10-B3:1
- 挿入:226 [Insert]: 前足外フレーム:1 ↔ ベアリングH　d6-D10-B3:2
- 挿入:227 [Insert] (-0.5 mm): 後ろ脚内フレーム２:1 ↔ 新型３脚最終段カム:2
- 挿入:228 [Insert] (6 mm): 脚モーターマウント:1 ↔ タミヤダンパー1:2
- メイト:99 [Mate]: 後ろ脚内内フレーム:1 ↔ タミヤダンパー1:2
- 挿入:229 [Insert]: 前足内フレーム:1 ↔ スペーサ　m3-l14:3
- 挿入:230 [Insert] (0.5 mm): 前足内フレーム:1 ↔ 新型３クランクアセンブリ:1
- 挿入:231 [Insert]: 中間内フレーム2:1 ↔ スペーサ　m3-l6:24
- 挿入:232 [Insert]: 中間内フレーム2:1 ↔ スペーサ　m3-l6:23
- 挿入:233 [Insert]: 中間内フレーム2:1 ↔ スペーサ　m3-l6:26
- 挿入:234 [Insert]: 中間内フレーム2:1 ↔ スペーサ　m3-l6:25
- 挿入:235 [Insert]: 中間内フレーム2:1 ↔ キャップボルトM3×8:27
- 挿入:236 [Insert]: 中間内フレーム2:1 ↔ キャップボルトM3×8:26
- 挿入:237 [Insert]: 前足ギアトレイン抑え:1 ↔ スペーサ　m3-l14:2
- メイト:100 [Mate]: 新型３脚最終段カム:4 ↔ フランジブッシュ　d12-14-F20:1
- 挿入:238 [Insert]: 前足ギアトレイン抑え:1 ↔ キャップボルトM3×20:2
- 挿入:239 [Insert]: 前足ギアトレイン抑え:1 ↔ キャップボルトM3×20:1
- 挿入:240 [Insert]: 前足ギアトレイン抑え:1 ↔ キャップボルトM3×20:3
- メイト:101 [Mate]: スペーサ　m3-l6:22 ↔ 新型４ウイング:1
- 挿入:241 [Insert]: キャップボルトM3×8:23 ↔ モーターマウントっぽい:1
- メイト:102 [Mate]: キャップボルトM3×8:25 ↔ モーターマウントっぽい:1
- 挿入:242 [Insert]: モーター(形だけ):1 ↔ モーターマウントっぽい:1
- 挿入:243 [Insert]: モーター(形だけ):2 ↔ モーターマウントっぽい:1
## Named parameters: d189_d187 = 0 mm, d191_d184 = 0 mm
